# Autodesk Inventor assembly: Battery Cart Storage Assembly
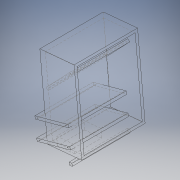
[picture p0: Inventor's stored thumbnail of the model, 180x180]
Saved by Autodesk Inventor 2018 (Build 220112000, 112)
## iProperties
Created: 2018-12-10
Part Number: Battery Cart Storage Assembly
Document SubType Name: Assembly
Designer: Gabriel
Author: Gabriel
## Documents named in this file (6)
- C:\Users\s-4009421\Downloads\Battery Cart Storage Assembly.iam
- C:\Users\s-4009421\Downloads\Cart Box.ipt
- C:\Users\s-4009421\Downloads\Cart Shelf.ipt
- C:\Users\s-4009421\Downloads\Bottom Bumper.ipt
- C:\Users\Gabriel\Downloads\BatteryModel.ipt
- C:\Users\s-4009421\Downloads\Battery Charger Representation.ipt
## Components (9 placed, 5 different names)
1. Cart Box:1 — Mate:1, Mate:2
2. Cart Shelf:2
3. Cart Shelf:3
4. Bottom Bumper:1
5. BatteryModel:1
6. BatteryModel:2
7. BatteryModel:3
8. Battery Charger Representation:1
9. Cart Shelf:4 — Mate:1, Mate:2
## Relationships (2: Mate 2)
- Mate:1: Cart Box:1 ↔ Cart Shelf:4
- Mate:2: Cart Box:1 ↔ Cart Shelf:4
